# Autodesk Inventor assembly: gripper_testing
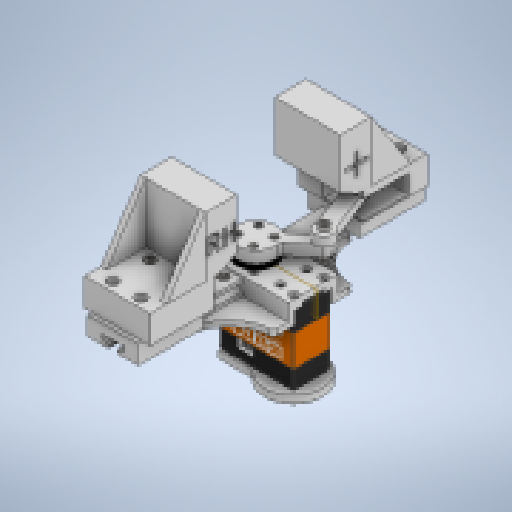
[picture p0: Inventor's stored thumbnail of the model, 512x512]
Saved by Autodesk Inventor 2024 (Build 280153000, 153)
## iProperties
Created: 2023-10-13
Part Number: gripper_testing
Document SubType Name: Assembly
Designer: 박동준
Author: 박동준
## Documents named in this file (17)
- C:\Users\박동준\OneDrive - 연세대학교 (Yonsei University)\바탕 화면\박동준\대학생할\로봇\Humanoid\7축 매니퓰레이터\하드웨어\rh_plus_7_axis_robot_arm_hardware\Assembly\3_Gripper.iam
- C:\Users\박동준\OneDrive - 연세대학교 (Yonsei University)\바탕 화면\박동준\대학생할\로봇\Humanoid\7축 매니퓰레이터\하드웨어\rh_plus_7_axis_robot_arm_hardware\Part\Frame\gripper\gripper.ipt
- C:\Users\박동준\OneDrive - 연세대학교 (Yonsei University)\바탕 화면\박동준\대학생할\로봇\Humanoid\7축 매니퓰레이터\하드웨어\rh_plus_7_axis_robot_arm_hardware\Part\Frame\gripper\gripper_base_frame.ipt
- C:\Users\박동준\OneDrive - 연세대학교 (Yonsei University)\바탕 화면\박동준\대학생할\로봇\Humanoid\7축 매니퓰레이터\하드웨어\rh_plus_7_axis_robot_arm_hardware\Part\Frame\axis_7_top_frame.ipt
- C:\Users\박동준\OneDrive - 연세대학교 (Yonsei University)\바탕 화면\박동준\대학생할\로봇\Humanoid\7축 매니퓰레이터\하드웨어\rh_plus_7_axis_robot_arm_hardware\Part\Frame\gripper\gripper_hand_connector.ipt
- C:\Users\박동준\OneDrive - 연세대학교 (Yonsei University)\바탕 화면\박동준\대학생할\로봇\Humanoid\7축 매니퓰레이터\하드웨어\rh_plus_7_axis_robot_arm_hardware\Part\Other Parts\lm_guide_cart.ipt
- C:\Users\박동준\OneDrive - 연세대학교 (Yonsei University)\바탕 화면\박동준\대학생할\로봇\Humanoid\7축 매니퓰레이터\하드웨어\rh_plus_7_axis_robot_arm_hardware\Part\Other Parts\lm_guide_rail.ipt
- C:\Users\박동준\OneDrive - 연세대학교 (Yonsei University)\바탕 화면\박동준\대학생할\로봇\Humanoid\7축 매니퓰레이터\하드웨어\rh_plus_7_axis_robot_arm_hardware\Part\HTD-45H, Horn\HTD-45H\HTD-45H.iam
- C:\Users\박동준\OneDrive - 연세대학교 (Yonsei University)\바탕 화면\박동준\대학생할\로봇\Humanoid\7축 매니퓰레이터\하드웨어\rh_plus_7_axis_robot_arm_hardware\Part\HTD-45H, Horn\Horn\Top Horn.ipt
- C:\Users\박동준\OneDrive - 연세대학교 (Yonsei University)\바탕 화면\박동준\대학생할\로봇\Humanoid\7축 매니퓰레이터\하드웨어\rh_plus_7_axis_robot_arm_hardware\Part\Bolt, Bearing, Nut, Washer\M2x10.ipt
- C:\Users\박동준\OneDrive - 연세대학교 (Yonsei University)\바탕 화면\박동준\대학생할\로봇\Humanoid\7축 매니퓰레이터\하드웨어\rh_plus_7_axis_robot_arm_hardware\Part\Bolt, Bearing, Nut, Washer\M3x8.ipt
- C:\Users\박동준\OneDrive - 연세대학교 (Yonsei University)\바탕 화면\박동준\대학생할\로봇\Humanoid\7축 매니퓰레이터\하드웨어\rh_plus_7_axis_robot_arm_hardware\Part\Frame\axis_7_bottom_frame.ipt
- C:\Users\박동준\OneDrive - 연세대학교 (Yonsei University)\바탕 화면\박동준\대학생할\로봇\Humanoid\7축 매니퓰레이터\하드웨어\rh_plus_7_axis_robot_arm_hardware\Part\Bolt, Bearing, Nut, Washer\2030 Teflon Sheet.ipt
- C:\Users\박동준\OneDrive - 연세대학교 (Yonsei University)\바탕 화면\박동준\대학생할\로봇\Humanoid\7축 매니퓰레이터\하드웨어\rh_plus_7_axis_robot_arm_hardware\Part\Bolt, Bearing, Nut, Washer\M2x6 Round Bolt.ipt
- C:\Users\박동준\OneDrive - 연세대학교 (Yonsei University)\Documents\Inventor\Content Center Files\R2024\en-US\BS 3692(1)\BS 3692 - M3(1).ipt
- C:\Users\박동준\OneDrive - 연세대학교 (Yonsei University)\Documents\Inventor\Content Center Files\R2024\en-US\CSN 02 1702  B\CSN 02 1702 - B 3.2.ipt
- C:\Users\박동준\OneDrive - 연세대학교 (Yonsei University)\바탕 화면\박동준\대학생할\로봇\Humanoid\7축 매니퓰레이터\하드웨어\rh_plus_7_axis_robot_arm_hardware\Part\Bolt, Bearing, Nut, Washer\M3x15.ipt
## Components (60 placed, 16 different names)
1. M3x8:1 — Rotational:13
2. M3x8:2 — Rotational:14
3. M3x8:3 — Rotational:16
4. M3x8:4 — Rotational:15
5. M3x8:6 — Rotational:19, Mate:76
6. M3x8:7 — Mate:65, Mate:66
7. M3x8:8 — Mate:61, Mate:62
8. M3x8:9 — Mate:63, Mate:64
9. M3x8:10 — Mate:55, Mate:56
10. M3x8:11 — Mate:59, Mate:60
11. M3x8:12 — Mate:57, Mate:58, Mate:27
12. M3x8:14 — Rotational:18, Mate:68
13. M3x15:1 — Mate:77, Mate:80, Mate:82, Mate:86, Mate:91
14. M3x15:2 — Mate:78, Mate:79, Mate:84, Mate:88, Mate:92
15. M2x6 Round Bolt:1 — Rigid:2
16. M2x6 Round Bolt:2 — Rigid:4
17. M2x6 Round Bolt:3 — Rigid:6
18. M2x6 Round Bolt:4 — Rigid:11
19. M2x6 Round Bolt:5 — Rigid:3
20. M2x6 Round Bolt:6 — Rigid:7
21. M2x6 Round Bolt:7 — Rigid:8
22. M2x6 Round Bolt:8 — Rigid:5
23. M2x6 Round Bolt:9 — Rigid:10
24. M2x6 Round Bolt:10 — Rigid:9
25. M2x6 Round Bolt:11 — Rigid:20
26. M2x6 Round Bolt:12 — Rigid:19
27. M2x6 Round Bolt:13 — Rigid:15
28. M2x6 Round Bolt:14 — Rigid:18
29. M2x6 Round Bolt:15 — Rigid:17
30. M2x6 Round Bolt:16 — Rigid:14
31. M2x6 Round Bolt:17 — Rigid:13
32. M2x6 Round Bolt:18 — Rigid:16
33. M2x10:1 — Rotational:1
34. M2x10:2 — Rotational:2
35. M2x10:3 — Rotational:4
36. M2x10:4 — Rotational:3
37. CSN 02 1702 B B 3.2:1 — Mate:69, Mate:91
38. CSN 02 1702 B B 3.2:2 — Mate:89, Mate:90
39. CSN 02 1702 B B 3.2:3 — Mate:71, Mate:92
40. CSN 02 1702 B B 3.2:4 — Mate:85, Mate:86
41. CSN 02 1702 B B 3.2:5 — Mate:67, Mate:68, Mate:73
42. CSN 02 1702 B B 3.2:6 — Mate:87, Mate:88
43. BS 3692 - Metric M3:1 — Mate:75, Mate:76, Mate:90
44. BS 3692 - Metric M3:2 — Mate:73, Mate:74
45. BS 3692 - Metric M3:3 — Mate:81, Mate:82, Mate:85
46. BS 3692 - Metric M3:4 — Mate:83, Mate:84
47. 2030 Teflon Sheet:1 — Rigid:12
48. gripper_base_frame:1 — Mate:3, Mate:4, Mate:5, Mate:24, Mate:43, Mate:25, Mate:30, Rotational:1, Rotational:2, Rotational:3, Rotational:4, Mate:81, Mate:83, Mate:87
49. axis_7_top_frame:1 — Mate:10, Mate:11, Angle:1, Mate:12, Mate:13, Mate:14, Mate:15, Mate:16, Mate:17, Rigid:13, Rigid:14, Rigid:15, Rigid:16, Rigid:17, Rigid:18, Rigid:19, Rigid:20
50. axis_7_bottom_frame:1 — Rigid:1, Rigid:2, Rigid:3, Rigid:4, Rigid:5, Rigid:6, Rigid:7, Rigid:8, Rigid:9, Rigid:10, Rigid:11, Rigid:12
51. HTD-45H:1 [sub-assembly] — Mate:1, Mate:2, Mate:10, Mate:11, Angle:1, Mate:49, Flush:2, Flush:3, Rigid:1
52. Top Horn:1 — Mate:1, Mate:2, Mate:3, Mate:4, Mate:5
53. gripper:1 — Angle:4, Mate:44, Mate:50, Mate:51, Rotational:19, Mate:61, Mate:62, Mate:63, Mate:64, Mate:65, Mate:66
54. gripper:2 — Mate:26, Mate:27, Mate:28, Mate:52, Rotational:18, Angle:5, Mate:55, Mate:56, Mate:57, Mate:58, Mate:59, Mate:60
55. gripper_hand_connector:1 — Mate:30, Mate:43, Mate:52, Mate:67, Mate:69, Mate:74, Mate:77, Mate:80
56. gripper_hand_connector:2 — Mate:24, Mate:25, Mate:51, Mate:71, Mate:75, Mate:78, Mate:79, Mate:89
57. lm_guide_cart:1 — Mate:18, Angle:2, Mate:19, Mate:26, Mate:28, Angle:5
58. lm_guide_cart:2 — Mate:20, Angle:3, Mate:21, Angle:4, Mate:44, Mate:50
59. lm_guide_rail:1 — Mate:12, Mate:13, Mate:14, Mate:18, Angle:2, Mate:19, Rotational:13, Rotational:14
60. lm_guide_rail:2 — Mate:15, Mate:16, Mate:17, Mate:20, Angle:3, Mate:21, Rotational:15, Rotational:16
## Relationships (102: Mate 65, WeldJoint 20, RevoluteJoint 10, Angle 5, Flush 2)
- Mate:1: HTD-45H:1 ↔ Top Horn:1
- Mate:2: HTD-45H:1 ↔ Top Horn:1
- Mate:3: gripper_base_frame:1 ↔ Top Horn:1
- Mate:4: gripper_base_frame:1 ↔ Top Horn:1
- Mate:5: gripper_base_frame:1 ↔ Top Horn:1
- Mate:10: axis_7_top_frame:1 ↔ HTD-45H:1
- Mate:11: axis_7_top_frame:1 ↔ HTD-45H:1
- Angle:1 (0 deg): axis_7_top_frame:1 ↔ HTD-45H:1
- Mate:12: axis_7_top_frame:1 ↔ lm_guide_rail:1
- Mate:13: axis_7_top_frame:1 ↔ lm_guide_rail:1
- Mate:14: axis_7_top_frame:1 ↔ lm_guide_rail:1
- Mate:15: axis_7_top_frame:1 ↔ lm_guide_rail:2
- Mate:16: axis_7_top_frame:1 ↔ lm_guide_rail:2
- Mate:17: axis_7_top_frame:1 ↔ lm_guide_rail:2
- Mate:18: lm_guide_cart:1 ↔ lm_guide_rail:1
- Angle:2 (0 deg): lm_guide_cart:1 ↔ lm_guide_rail:1
- Mate:19: lm_guide_cart:1 ↔ lm_guide_rail:1
- Mate:20: lm_guide_cart:2 ↔ lm_guide_rail:2
- Angle:3 (0 deg): lm_guide_cart:2 ↔ lm_guide_rail:2
- Mate:21: lm_guide_cart:2 ↔ lm_guide_rail:2
- Mate:24 (0.5 mm): gripper_base_frame:1 ↔ gripper_hand_connector:2
- Mate:43 (0.5 mm): gripper_base_frame:1 ↔ gripper_hand_connector:1
- Mate:25: gripper_base_frame:1 ↔ gripper_hand_connector:2
- Angle:4 (0 deg): gripper:1 ↔ lm_guide_cart:2
- Mate:26: gripper:2 ↔ lm_guide_cart:1
- Mate:27: M3x8:12 ↔ gripper:2
- Mate:28: gripper:2 ↔ lm_guide_cart:1
- Mate:30: gripper_base_frame:1 ↔ gripper_hand_connector:1
- Rotational:1 [RevoluteJoint]: M2x10:1 ↔ gripper_base_frame:1
- Rotational:2 [RevoluteJoint]: M2x10:2 ↔ gripper_base_frame:1
- Rotational:3 [RevoluteJoint]: M2x10:4 ↔ gripper_base_frame:1
- Rotational:4 [RevoluteJoint]: M2x10:3 ↔ gripper_base_frame:1
- Rotational:13 [RevoluteJoint]: M3x8:1 ↔ lm_guide_rail:1
- Rotational:14 [RevoluteJoint]: M3x8:2 ↔ lm_guide_rail:1
- Rotational:15 [RevoluteJoint]: M3x8:4 ↔ lm_guide_rail:2
- Mate:44: gripper:1 ↔ lm_guide_cart:2
- Rotational:16 [RevoluteJoint]: M3x8:3 ↔ lm_guide_rail:2
- Mate:49: HTD-45H:1
- Flush:2: HTD-45H:1
- Flush:3: HTD-45H:1
- Rigid:1 [WeldJoint]: axis_7_bottom_frame:1 ↔ HTD-45H:1
- Rigid:2 [WeldJoint]: M2x6 Round Bolt:1 ↔ axis_7_bottom_frame:1
- Rigid:3 [WeldJoint]: M2x6 Round Bolt:5 ↔ axis_7_bottom_frame:1
- Rigid:4 [WeldJoint]: M2x6 Round Bolt:2 ↔ axis_7_bottom_frame:1
- Rigid:5 [WeldJoint]: M2x6 Round Bolt:8 ↔ axis_7_bottom_frame:1
- Rigid:6 [WeldJoint]: M2x6 Round Bolt:3 ↔ axis_7_bottom_frame:1
- Rigid:7 [WeldJoint]: M2x6 Round Bolt:6 ↔ axis_7_bottom_frame:1
- Rigid:8 [WeldJoint]: M2x6 Round Bolt:7 ↔ axis_7_bottom_frame:1
- Rigid:9 [WeldJoint]: M2x6 Round Bolt:10 ↔ axis_7_bottom_frame:1
- Rigid:10 [WeldJoint]: M2x6 Round Bolt:9 ↔ axis_7_bottom_frame:1
- Rigid:11 [WeldJoint]: M2x6 Round Bolt:4 ↔ axis_7_bottom_frame:1
- Rigid:12 [WeldJoint]: 2030 Teflon Sheet:1 ↔ axis_7_bottom_frame:1
- Rigid:13 [WeldJoint]: M2x6 Round Bolt:17 ↔ axis_7_top_frame:1
- Rigid:14 [WeldJoint]: M2x6 Round Bolt:16 ↔ axis_7_top_frame:1
- Rigid:15 [WeldJoint]: M2x6 Round Bolt:13 ↔ axis_7_top_frame:1
- Rigid:16 [WeldJoint]: M2x6 Round Bolt:18 ↔ axis_7_top_frame:1
- Rigid:17 [WeldJoint]: M2x6 Round Bolt:15 ↔ axis_7_top_frame:1
- Rigid:18 [WeldJoint]: M2x6 Round Bolt:14 ↔ axis_7_top_frame:1
- Rigid:19 [WeldJoint]: M2x6 Round Bolt:12 ↔ axis_7_top_frame:1
- Rigid:20 [WeldJoint]: M2x6 Round Bolt:11 ↔ axis_7_top_frame:1
- Mate:50: gripper:1 ↔ lm_guide_cart:2
- Mate:51: gripper:1 ↔ gripper_hand_connector:2
- Mate:52: gripper:2 ↔ gripper_hand_connector:1
- Rotational:18 [RevoluteJoint]: M3x8:14 ↔ gripper:2
- Rotational:19 [RevoluteJoint]: M3x8:6 ↔ gripper:1
- Angle:5 (0 deg): gripper:2 ↔ lm_guide_cart:1
- Mate:55: M3x8:10 ↔ gripper:2
- Mate:56: M3x8:10 ↔ gripper:2
- Mate:57: M3x8:12 ↔ gripper:2
- Mate:58: M3x8:12 ↔ gripper:2
- Mate:59: M3x8:11 ↔ gripper:2
- Mate:60: M3x8:11 ↔ gripper:2
- Mate:61: M3x8:8 ↔ gripper:1
- Mate:62: M3x8:8 ↔ gripper:1
- Mate:63: M3x8:9 ↔ gripper:1
- Mate:64: M3x8:9 ↔ gripper:1
- Mate:65: M3x8:7 ↔ gripper:1
- Mate:66: M3x8:7 ↔ gripper:1
- Mate:67: CSN 02 1702 B B 3.2:5 ↔ gripper_hand_connector:1
- Mate:68: M3x8:14 ↔ CSN 02 1702 B B 3.2:5
- Mate:69: CSN 02 1702 B B 3.2:1 ↔ gripper_hand_connector:1
- Mate:71: CSN 02 1702 B B 3.2:3 ↔ gripper_hand_connector:2
- Mate:73: CSN 02 1702 B B 3.2:5 ↔ BS 3692 - Metric M3:2
- Mate:74: BS 3692 - Metric M3:2 ↔ gripper_hand_connector:1
- Mate:75 (0.5 mm): BS 3692 - Metric M3:1 ↔ gripper_hand_connector:2
- Mate:76: M3x8:6 ↔ BS 3692 - Metric M3:1
- Mate:77: M3x15:1 ↔ gripper_hand_connector:1
- Mate:78: M3x15:2 ↔ gripper_hand_connector:2
- Mate:79: M3x15:2 ↔ gripper_hand_connector:2
- Mate:80: M3x15:1 ↔ gripper_hand_connector:1
- Mate:81 (0.5 mm): BS 3692 - Metric M3:3 ↔ gripper_base_frame:1
- Mate:82: M3x15:1 ↔ BS 3692 - Metric M3:3
- Mate:83 (0.5 mm): BS 3692 - Metric M3:4 ↔ gripper_base_frame:1
- Mate:84: M3x15:2 ↔ BS 3692 - Metric M3:4
- Mate:85: CSN 02 1702 B B 3.2:4 ↔ BS 3692 - Metric M3:3
- Mate:86: M3x15:1 ↔ CSN 02 1702 B B 3.2:4
- Mate:87: CSN 02 1702 B B 3.2:6 ↔ gripper_base_frame:1
- Mate:88: M3x15:2 ↔ CSN 02 1702 B B 3.2:6
- Mate:89: CSN 02 1702 B B 3.2:2 ↔ gripper_hand_connector:2
- Mate:90: CSN 02 1702 B B 3.2:2 ↔ BS 3692 - Metric M3:1
- Mate:91: M3x15:1 ↔ CSN 02 1702 B B 3.2:1
- Mate:92: M3x15:2 ↔ CSN 02 1702 B B 3.2:3
